# Autodesk Inventor assembly: Limit switch
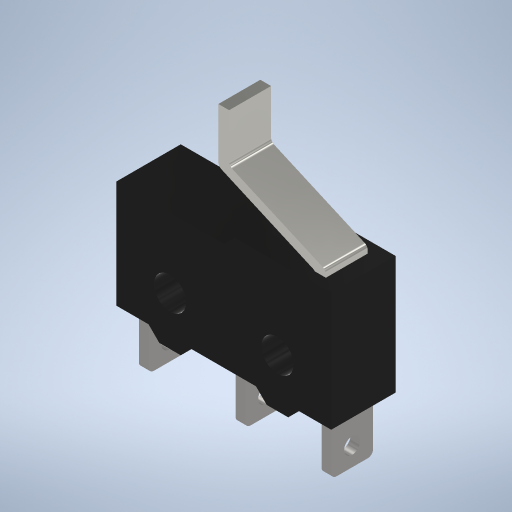
[picture p0: Inventor's stored thumbnail of the model, 512x512]
Saved by Autodesk Inventor 2023 (Build 270158000, 158)
## iProperties
Created: 2023-12-14
Part Number: Limit switch
Document SubType Name: Assembly
Designer: User
Author: User
## Documents named in this file (4)
- G:\Downloads\INVENTOR WEIGH SCALE\Limit switch.iam
- G:\Downloads\INVENTOR WEIGH SCALE\Limit switch body.ipt
- G:\Downloads\INVENTOR WEIGH SCALE\Limit switch pin.ipt
- G:\Downloads\INVENTOR WEIGH SCALE\Limit switch sheet.ipt
## Components (5 placed, 3 different names)
1. Limit switch body:1 — Mate:1, Mate:2, Mate:3, Mate:4, Mate:5, Mate:6, Mate:7, Mate:8, Mate:9, Mate:10, Mate:11, Mate:12, Mate:13
2. Limit switch pin:1 — Mate:1, Mate:2, Mate:3
3. Limit switch pin:2 — Mate:4, Mate:5, Mate:6
4. Limit switch pin:3 — Mate:7, Mate:8, Mate:9
5. Limit switch sheet:1 — Mate:10, Mate:11, Mate:12, Mate:13
## Relationships (13: Mate 13)
- Mate:1: Limit switch body:1 ↔ Limit switch pin:1
- Mate:2: Limit switch body:1 ↔ Limit switch pin:1
- Mate:3: Limit switch body:1 ↔ Limit switch pin:1
- Mate:4: Limit switch body:1 ↔ Limit switch pin:2
- Mate:5: Limit switch body:1 ↔ Limit switch pin:2
- Mate:6: Limit switch body:1 ↔ Limit switch pin:2
- Mate:7: Limit switch body:1 ↔ Limit switch pin:3
- Mate:8: Limit switch body:1 ↔ Limit switch pin:3
- Mate:9: Limit switch body:1 ↔ Limit switch pin:3
- Mate:10: Limit switch body:1 ↔ Limit switch sheet:1
- Mate:11: Limit switch body:1 ↔ Limit switch sheet:1
- Mate:12: Limit switch body:1 ↔ Limit switch sheet:1
- Mate:13: Limit switch body:1 ↔ Limit switch sheet:1
